# Autodesk Inventor assembly: Рама
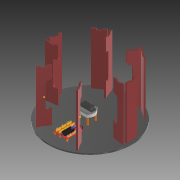
[picture p0: Inventor's stored thumbnail of the model, 180x180]
Saved by Autodesk Inventor 2022 (Build 260153000, 153)
## iProperties
Created: 2025-01-23
Part Number: Рама
Document SubType Name: Assembly
Designer: Ivan
Mass: 1271.55 g
Surface Area: 4932.14 cm^2
Volume: 1271.55 cm^3
Density: 1 g/cm^3
Author: Ivan
Title: Рама
## Documents named in this file (7)
- E:\Предпроф 2025\Shoter_1_ZIP\Рама.iam
- E:\Предпроф 2025\Shoter_1_ZIP\Основание_нижнее.ipt
- E:\Предпроф 2025\Shoter_1_ZIP\Планка боковая.ipt
- E:\Предпроф 2025\Shoter_1_ZIP\Планка_опорная.ipt
- E:\Предпроф 2025\Shoter_1_ZIP\Сборка_сервопривода.iam
- E:\Предпроф 2025\Shoter_1_ZIP\Стойка м3х10.ipt
- E:\Предпроф 2025\Shoter_1_ZIP\Keyestudio CNC Shield Arduino Nano.ipt
## Components (18 placed, 6 different names)
1. Основание_нижнее:1 — Совмещение:1, Совмещение:2, Заподлицо:1, Совмещение:3, Совмещение:4, Совмещение:5, Заподлицо:2, Совмещение:6, Совмещение:7, Совмещение:8, Совмещение:9, Совмещение:10, Совмещение:11, Совмещение:12, Совмещение:13, Заподлицо:3, Заподлицо:4, Заподлицо:5, Заподлицо:6, Заподлицо:7, Совмещение:14, Совмещение:15, Заподлицо:8, Совмещение:16, Совмещение:17, Совмещение:18, Заподлицо:9, Совмещение:19, Совмещение:20, Совмещение:21, Совмещение:22, Заподлицо:10, Заподлицо:11, Совмещение:23, Совмещение:24, Совмещение:25, Совмещение:26, Совмещение:27, Совмещение:28, Совмещение:29, Совмещение:30, Совмещение:31
2. Планка боковая:1 — Совмещение:1, Совмещение:2, Заподлицо:1
3. Планка боковая:2 — Совмещение:3, Заподлицо:7, Совмещение:14
4. Планка боковая:3 — Совмещение:4, Совмещение:13, Заподлицо:6
5. Планка боковая:4 — Совмещение:7, Совмещение:12, Заподлицо:5
6. Планка боковая:5 — Совмещение:8, Совмещение:11, Заподлицо:4
7. Планка боковая:6 — Совмещение:9, Совмещение:10, Заподлицо:3
8. Планка_опорная:1 — Совмещение:15, Заподлицо:8, Совмещение:16
9. Планка_опорная:2 — Совмещение:17, Совмещение:18, Заподлицо:9
10. Планка_опорная:3 — Совмещение:19, Совмещение:20, Заподлицо:11
11. Планка_опорная:4 — Совмещение:21, Совмещение:22, Заподлицо:10
12. Сборка_сервопривода:1 [sub-assembly] — Совмещение:23, Совмещение:24, Совмещение:25, Угол:1
13. Стойка м3х10:1 — Совмещение:27, Заподлицо:12, Заподлицо:13, Совмещение:32
14. Стойка м3х10:2 — Совмещение:28, Заподлицо:15
15. Стойка м3х10:3 — Совмещение:29, Заподлицо:14, Заподлицо:15, Совмещение:31
16. Стойка м3х10:4 — Совмещение:26, Заподлицо:12
17. Стойка м3х10:5 — Совмещение:30, Заподлицо:13, Заподлицо:14, Совмещение:33
18. Keyestudio CNC Shield Arduino Nano:1 — Совмещение:32, Совмещение:33, Угол:1
## Relationships (49: Mate 33, Flush 15, Angle 1)
- Совмещение:1 [Mate]: Основание_нижнее:1 ↔ Планка боковая:1
- Совмещение:2 [Mate]: Основание_нижнее:1 ↔ Планка боковая:1
- Заподлицо:1 [Flush]: Основание_нижнее:1 ↔ Планка боковая:1
- Совмещение:3 [Mate]: Основание_нижнее:1 ↔ Планка боковая:2
- Совмещение:4 [Mate]: Основание_нижнее:1 ↔ Планка боковая:3
- Совмещение:5 [Mate]: Основание_нижнее:1
- Заподлицо:2 [Flush]: Основание_нижнее:1
- Совмещение:6 [Mate]: Основание_нижнее:1
- Совмещение:7 [Mate]: Основание_нижнее:1 ↔ Планка боковая:4
- Совмещение:8 [Mate]: Основание_нижнее:1 ↔ Планка боковая:5
- Совмещение:9 [Mate]: Основание_нижнее:1 ↔ Планка боковая:6
- Совмещение:10 [Mate]: Основание_нижнее:1 ↔ Планка боковая:6
- Совмещение:11 [Mate]: Основание_нижнее:1 ↔ Планка боковая:5
- Совмещение:12 [Mate]: Основание_нижнее:1 ↔ Планка боковая:4
- Совмещение:13 [Mate]: Основание_нижнее:1 ↔ Планка боковая:3
- Заподлицо:3 [Flush]: Основание_нижнее:1 ↔ Планка боковая:6
- Заподлицо:4 [Flush]: Основание_нижнее:1 ↔ Планка боковая:5
- Заподлицо:5 [Flush]: Основание_нижнее:1 ↔ Планка боковая:4
- Заподлицо:6 [Flush]: Основание_нижнее:1 ↔ Планка боковая:3
- Заподлицо:7 [Flush]: Основание_нижнее:1 ↔ Планка боковая:2
- Совмещение:14 [Mate]: Основание_нижнее:1 ↔ Планка боковая:2
- Совмещение:15 [Mate]: Основание_нижнее:1 ↔ Планка_опорная:1
- Заподлицо:8 [Flush]: Основание_нижнее:1 ↔ Планка_опорная:1
- Совмещение:16 [Mate]: Основание_нижнее:1 ↔ Планка_опорная:1
- Совмещение:17 [Mate]: Основание_нижнее:1 ↔ Планка_опорная:2
- Совмещение:18 [Mate]: Основание_нижнее:1 ↔ Планка_опорная:2
- Заподлицо:9 [Flush]: Основание_нижнее:1 ↔ Планка_опорная:2
- Совмещение:19 [Mate]: Основание_нижнее:1 ↔ Планка_опорная:3
- Совмещение:20 [Mate]: Основание_нижнее:1 ↔ Планка_опорная:3
- Совмещение:21 [Mate]: Основание_нижнее:1 ↔ Планка_опорная:4
- Совмещение:22 [Mate]: Основание_нижнее:1 ↔ Планка_опорная:4
- Заподлицо:10 [Flush]: Основание_нижнее:1 ↔ Планка_опорная:4
- Заподлицо:11 [Flush]: Основание_нижнее:1 ↔ Планка_опорная:3
- Совмещение:23 [Mate]: Основание_нижнее:1 ↔ Сборка_сервопривода:1
- Совмещение:24 [Mate]: Основание_нижнее:1 ↔ Сборка_сервопривода:1
- Совмещение:25 [Mate]: Основание_нижнее:1 ↔ Сборка_сервопривода:1
- Совмещение:26 [Mate]: Основание_нижнее:1 ↔ Стойка м3х10:4
- Совмещение:27 [Mate]: Основание_нижнее:1 ↔ Стойка м3х10:1
- Совмещение:28 [Mate]: Основание_нижнее:1 ↔ Стойка м3х10:2
- Совмещение:29 [Mate]: Основание_нижнее:1 ↔ Стойка м3х10:3
- Совмещение:30 [Mate]: Основание_нижнее:1 ↔ Стойка м3х10:5
- Заподлицо:12 [Flush]: Стойка м3х10:1 ↔ Стойка м3х10:4
- Заподлицо:13 [Flush]: Стойка м3х10:1 ↔ Стойка м3х10:5
- Заподлицо:14 [Flush]: Стойка м3х10:3 ↔ Стойка м3х10:5
- Заподлицо:15 [Flush]: Стойка м3х10:2 ↔ Стойка м3х10:3
- Совмещение:31 [Mate]: Основание_нижнее:1 ↔ Стойка м3х10:3
- Совмещение:32 [Mate]: Стойка м3х10:1 ↔ Keyestudio CNC Shield Arduino Nano:1
- Совмещение:33 [Mate]: Стойка м3х10:5 ↔ Keyestudio CNC Shield Arduino Nano:1
- Угол:1 [Angle] (0 deg): Сборка_сервопривода:1 ↔ Keyestudio CNC Shield Arduino Nano:1
